# Autodesk Inventor assembly: ShakerAssembly
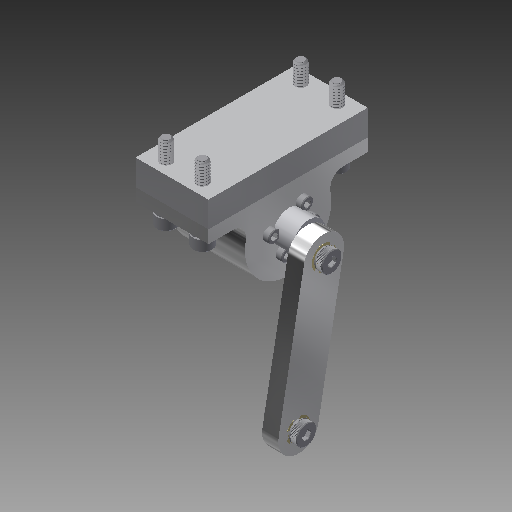
[picture p0: Inventor's stored thumbnail of the model, 512x512]
Saved by Autodesk Inventor 2017 (Build 210142000, 142)
## iProperties
Created: 2017-02-08
Part Number: ShakerAssembly
Document SubType Name: Assembly
Designer: Joseph
Author: Joseph
## Documents named in this file (11)
- C:\UMD\BPP\ROCKSAT X\STAR\CAD\Mechanical\Full payload assembly\Subsystems\Shaker\ShakerAssembly.iam
- C:\UMD\BPP\ROCKSAT X\STAR\CAD\Mechanical\Full payload assembly\Subsystems\Shaker\Motor.ipt
- C:\UMD\BPP\ROCKSAT X\STAR\CAD\Mechanical\Full payload assembly\Subsystems\Shaker\Motor Arm.ipt
- C:\UMD\BPP\ROCKSAT X\STAR\CAD\Mechanical\Full payload assembly\Subsystems\Shaker\Linkage.ipt
- C:\UMD\BPP\ROCKSAT X\STAR\CAD\Mechanical\Full payload assembly\Subsystems\Shaker\Motor Holder.ipt
- C:\UMD\BPP\ROCKSAT X\STAR\CAD\Mechanical\Full payload assembly\Subsystems\Shaker\Oil-Sleeve Bearing.ipt
- C:\UMD\BPP\ROCKSAT X\STAR\CAD\Mechanical\Full payload assembly\Subsystems\Fasteners\M1.6x.35mm 4mm Socket Screw.ipt
- C:\UMD\BPP\ROCKSAT X\STAR\CAD\Mechanical\Full payload assembly\Subsystems\Fasteners\M2x.4mm 4mm Screw .ipt
- C:\UMD\BPP\ROCKSAT X\STAR\CAD\Mechanical\Full payload assembly\Subsystems\Shaker\MotorMountSpacer.ipt
- C:\UMD\BPP\ROCKSAT X\STAR\CAD\Mechanical\Full payload assembly\Subsystems\Fasteners\Num4 Narrow Split Washer.ipt
- C:\UMD\BPP\ROCKSAT X\STAR\CAD\Mechanical\Full payload assembly\Subsystems\Fasteners\4-40 .625in Socket Screw.ipt
## Components (22 placed, 10 different names)
1. Motor:1 — Insert:1, Insert:2
2. Motor:1 — Insert:1, Insert:2, Rotational:1, Mate:2, Mate:3, Mate:4, Mate:5
3. Motor Arm:1 — Rotational:1, Mate:8, Mate:21
4. Linkage:1 — Mate:6, Flush:1, Flush:2, Mate:7, Mate:8, Mate:17, Mate:18
5. Motor Holder:1 — Mate:2, Mate:3, Mate:4, Mate:5, Mate:9, Mate:10, Mate:11, Mate:12, Mate:13, Mate:14, Mate:15, Mate:16, Mate:22, Flush:3, Flush:4, Mate:23, Mate:24, Mate:25, Mate:26, Mate:27, Mate:28, Mate:29, Mate:30, Mate:31, Mate:32
6. Oil-Sleeve Bearing:1 — Flush:2, Mate:7, Mate:19
7. Oil-Sleeve Bearing:2 — Mate:6, Flush:1, Mate:20
8. M1.6x.35mm 4mm Socket Screw:1 — Mate:9, Mate:16
9. M1.6x.35mm 4mm Socket Screw:2 — Mate:10, Mate:14
10. M1.6x.35mm 4mm Socket Screw:3 — Mate:11, Mate:13
11. M1.6x.35mm 4mm Socket Screw:4 — Mate:12, Mate:15
12. M2x.4mm 4mm Screw :1 — Mate:18, Mate:19, Mate:21
13. M2x.4mm 4mm Screw :2 — Mate:17, Mate:20
14. MotorMountSpacer:1 — Mate:22, Flush:3, Flush:4
15. Num4 Narrow Split Washer:1 — Mate:24, Mate:30, Mate:33, Mate:35
16. Num4 Narrow Split Washer:2 — Mate:23, Mate:29, Mate:34, Mate:36
17. Num4 Narrow Split Washer:3 — Mate:25, Mate:27, Mate:37
18. Num4 Narrow Split Washer:4 — Mate:26, Mate:28, Mate:38
19. 4-40 .625in Socket Screw:1 — Mate:31, Mate:37
20. 4-40 .625in Socket Screw:2 — Mate:32, Mate:38
21. 4-40 .625in Socket Screw:3 — Mate:33, Mate:35
22. 4-40 .625in Socket Screw:4 — Mate:34, Mate:36
## Relationships (44: Mate 37, Flush 4, Insert 2, RevoluteJoint 1)
- Insert:1: Motor:1
- Insert:2: Motor:1
- Rotational:1 [RevoluteJoint]: Motor:1 ↔ Motor Arm:1
- Mate:2: Motor:1 ↔ Motor Holder:1
- Mate:3: Motor:1 ↔ Motor Holder:1
- Mate:4: Motor:1 ↔ Motor Holder:1
- Mate:5: Motor:1 ↔ Motor Holder:1
- Mate:6: Linkage:1 ↔ Oil-Sleeve Bearing:2
- Flush:1: Linkage:1 ↔ Oil-Sleeve Bearing:2
- Flush:2: Linkage:1 ↔ Oil-Sleeve Bearing:1
- Mate:7: Linkage:1 ↔ Oil-Sleeve Bearing:1
- Mate:8: Motor Arm:1 ↔ Linkage:1
- Mate:9: Motor Holder:1 ↔ M1.6x.35mm 4mm Socket Screw:1
- Mate:10: Motor Holder:1 ↔ M1.6x.35mm 4mm Socket Screw:2
- Mate:11: Motor Holder:1 ↔ M1.6x.35mm 4mm Socket Screw:3
- Mate:12: Motor Holder:1 ↔ M1.6x.35mm 4mm Socket Screw:4
- Mate:13: Motor Holder:1 ↔ M1.6x.35mm 4mm Socket Screw:3
- Mate:14: Motor Holder:1 ↔ M1.6x.35mm 4mm Socket Screw:2
- Mate:15: Motor Holder:1 ↔ M1.6x.35mm 4mm Socket Screw:4
- Mate:16: Motor Holder:1 ↔ M1.6x.35mm 4mm Socket Screw:1
- Mate:17: Linkage:1 ↔ M2x.4mm 4mm Screw :2
- Mate:18: Linkage:1 ↔ M2x.4mm 4mm Screw :1
- Mate:19: Oil-Sleeve Bearing:1 ↔ M2x.4mm 4mm Screw :1
- Mate:20: Oil-Sleeve Bearing:2 ↔ M2x.4mm 4mm Screw :2
- Mate:21: Motor Arm:1 ↔ M2x.4mm 4mm Screw :1
- Mate:22: Motor Holder:1 ↔ MotorMountSpacer:1
- Flush:3: Motor Holder:1 ↔ MotorMountSpacer:1
- Flush:4: Motor Holder:1 ↔ MotorMountSpacer:1
- Mate:23: Motor Holder:1 ↔ Num4 Narrow Split Washer:2
- Mate:24: Motor Holder:1 ↔ Num4 Narrow Split Washer:1
- Mate:25: Motor Holder:1 ↔ Num4 Narrow Split Washer:3
- Mate:26: Motor Holder:1 ↔ Num4 Narrow Split Washer:4
- Mate:27: Motor Holder:1 ↔ Num4 Narrow Split Washer:3
- Mate:28: Motor Holder:1 ↔ Num4 Narrow Split Washer:4
- Mate:29: Motor Holder:1 ↔ Num4 Narrow Split Washer:2
- Mate:30: Motor Holder:1 ↔ Num4 Narrow Split Washer:1
- Mate:31: Motor Holder:1 ↔ 4-40 .625in Socket Screw:1
- Mate:32: Motor Holder:1 ↔ 4-40 .625in Socket Screw:2
- Mate:33: Num4 Narrow Split Washer:1 ↔ 4-40 .625in Socket Screw:3
- Mate:34: Num4 Narrow Split Washer:2 ↔ 4-40 .625in Socket Screw:4
- Mate:35: Num4 Narrow Split Washer:1 ↔ 4-40 .625in Socket Screw:3
- Mate:36: Num4 Narrow Split Washer:2 ↔ 4-40 .625in Socket Screw:4
- Mate:37: Num4 Narrow Split Washer:3 ↔ 4-40 .625in Socket Screw:1
- Mate:38: Num4 Narrow Split Washer:4 ↔ 4-40 .625in Socket Screw:2
